# Autodesk Inventor assembly: assenbly
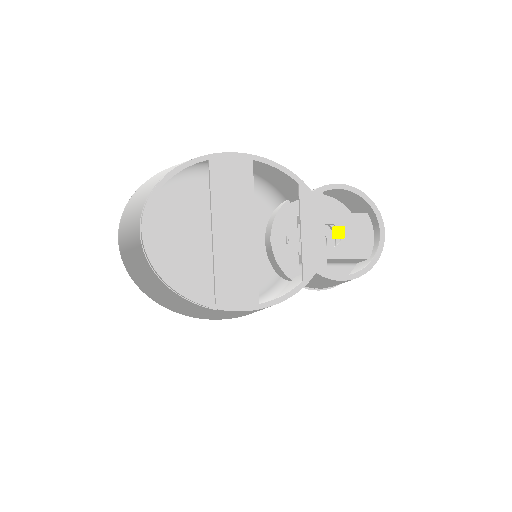
[picture p0: Inventor's stored thumbnail of the model, 512x512]
Saved by Autodesk Inventor 2025.2 (Build 292293000, 293)
## iProperties
Created: 2025-06-18
Part Number: assenbly
Document SubType Name: Assembly
Designer: joseph
Author: joseph
## Documents named in this file (7)
- C:\Users\2001j\OneDrive - inha.edu\2025 식사보조기구 모델링\assenbly.iam
- C:\Users\2001j\OneDrive - inha.edu\2025 식사보조기구 모델링\arm_1 (only rotate).ipt
- C:\Users\2001j\OneDrive - inha.edu\2025 식사보조기구 모델링\Plate Body.ipt
- C:\Users\2001j\OneDrive - inha.edu\2025 식사보조기구 모델링\arm_2 (first arm).ipt
- C:\Users\2001j\OneDrive - inha.edu\2025 식사보조기구 모델링\arm_3 (second arm).ipt
- C:\Users\2001j\OneDrive - inha.edu\2025 식사보조기구 모델링\end arm_1.ipt
- C:\Users\2001j\OneDrive - inha.edu\2025 식사보조기구 모델링\end arm_2.ipt
## Components (6 placed, 6 different names)
1. arm_1 (only rotate):1 — 회전:1, 회전:2
2. Plate Body:1 — 회전:1
3. arm_2 (first arm):1 — 회전:2
4. arm_3 (second arm):1
5. end arm_1:1
6. end arm_2:1
## Relationships (2: RevoluteJoint 2)
- 회전:1 [RevoluteJoint]: arm_1 (only rotate):1 ↔ Plate Body:1
- 회전:2 [RevoluteJoint]: arm_1 (only rotate):1 ↔ arm_2 (first arm):1
